# Autodesk Inventor assembly: Motor_in_Enclosure
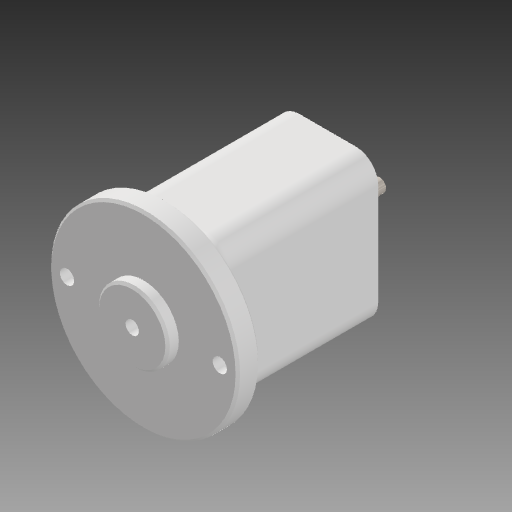
[picture p0: Inventor's stored thumbnail of the model, 512x512]
Saved by Autodesk Inventor 2024 (Build 280153000, 153)
## iProperties
Created: 2024-03-16
Part Number: Motor_in_Enclosure
Document SubType Name: Assembly
Designer: Faber
Author: Faber
## Documents named in this file (3)
- C:\Users\Bluex\Documents\GitHub\Autonome_Robotter\3D_inventor_robor_hånd\Motor_in_Enclosure.iam
- C:\Users\Bluex\Documents\GitHub\Autonome_Robotter\3D_inventor_robor_hånd\Motor_Enclosure.ipt
- C:\Users\Bluex\Documents\GitHub\Autonome_Robotter\3D_inventor_robor_hånd\Motor-HG37-300-AB-00\3D\HG37-300-AB-00\HG37-300-AB-00.iam
## Components (2 placed, 2 different names)
1. Motor_Enclosure:1 — Mate:1, Flush:1
2. HG37-300-AB-00:1 [sub-assembly] — Mate:1, Flush:1
## Relationships (2: Mate 1, Flush 1)
- Mate:1: Motor_Enclosure:1 ↔ HG37-300-AB-00:1
- Flush:1: Motor_Enclosure:1 ↔ HG37-300-AB-00:1
